# Autodesk Inventor assembly: focus_m12_n12_f=6.0lam_to_14.0lam_step=2.0lam_assembly
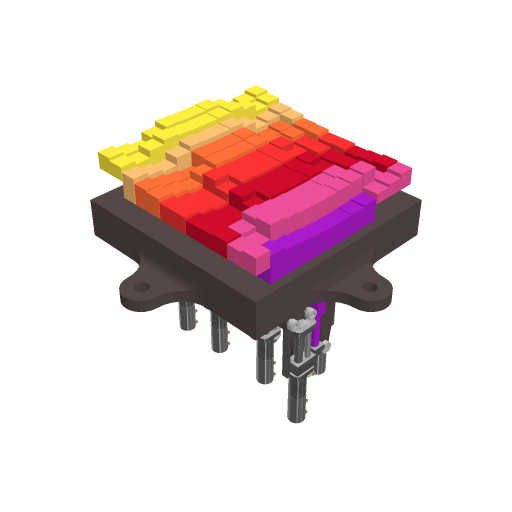
[picture p0: Inventor's stored thumbnail of the model, 512x512]
Saved by Autodesk Inventor 2023 (Build 270158000, 158)
## iProperties
Created: 2022-08-15
Part Number: focus_m12_n12_f=6.0lam_to_14.0lam_step=2.0lam_assembly
Document SubType Name: Assembly
Designer: James
Author: James
## Documents named in this file (14)
- C:\Users\James\OneDrive - University College London\Activation of Metasurface\Ben Motors\SSM_assembly\focus_m12_n12_f=6.0lam_to_14.0lam_step=2.0lam_assembly.iam
- C:\Users\James\OneDrive - University College London\Activation of Metasurface\Ben Motors\SSM_assembly\seg_1.ipt
- C:\Users\James\OneDrive - University College London\Activation of Metasurface\Ben Motors\SSM_assembly\seg_2.ipt
- C:\Users\James\OneDrive - University College London\Activation of Metasurface\Ben Motors\SSM_assembly\seg_3.ipt
- C:\Users\James\OneDrive - University College London\Activation of Metasurface\Ben Motors\SSM_assembly\seg_4.ipt
- C:\Users\James\OneDrive - University College London\Activation of Metasurface\Ben Motors\SSM_assembly\seg_5.ipt
- C:\Users\James\OneDrive - University College London\Activation of Metasurface\Ben Motors\SSM_assembly\seg_6.ipt
- C:\Users\James\OneDrive - University College London\Activation of Metasurface\Ben Motors\SSM_assembly\seg_7.ipt
- C:\Users\James\OneDrive - University College London\Activation of Metasurface\Ben Motors\SSM_assembly\jig.iam
- C:\Users\James\OneDrive - University College London\Activation of Metasurface\Ben Motors\SSM_assembly\motor_lowest.ipt
- C:\Users\James\OneDrive - University College London\Activation of Metasurface\Ben Motors\SSM_assembly\motor_mid.ipt
- C:\Users\James\OneDrive - University College London\Activation of Metasurface\Ben Motors\SSM_assembly\motor_highest.ipt
- C:\Users\James\OneDrive - University College London\Activation of Metasurface\Ben Motors\SSM_assembly\M1.4 Hex Screw v3.ipt
- C:\Users\James\OneDrive - University College London\Activation of Metasurface\Ben Motors\SSM_assembly\Nut M1.4 v3.ipt
## Components (57 placed, 13 different names)
1. jig:1 [sub-assembly] — Mate:16, Flush:8, Mate:19, Mate:20, Mate:24, Mate:25, Mate:26, Mate:28, Flush:9, Mate:29, Flush:10, Flush:11, Flush:12, Flush:13, Flush:14, Flush:15, Flush:16, Flush:17, Flush:18, Flush:19, Flush:20, Flush:21, Flush:22, Flush:23, Mate:90, Mate:91, Mate:126, Mate:127
2. motor_highest:1 — Mate:28, Flush:10, Flush:17, Mate:45, Mate:46, Mate:47, Mate:48, Mate:49
3. motor_mid:1 — Mate:19, Flush:15, Flush:22, Mate:74, Mate:75, Mate:76, Mate:77, Mate:78, Mate:79
4. motor_mid:2 — Mate:20, Flush:13, Flush:21, Mate:62, Mate:63, Mate:64, Mate:65, Mate:66, Mate:67
5. motor_mid:3 — Mate:24, Flush:14, Flush:19, Mate:68, Mate:69, Mate:70, Mate:71, Mate:72, Mate:73
6. motor_mid:4 — Mate:25, Flush:12, Flush:18, Mate:56, Mate:57, Mate:58, Mate:59, Mate:60, Mate:61
7. motor_mid:5 — Mate:26, Flush:11, Flush:20, Mate:50, Mate:51, Mate:52, Mate:53, Mate:54, Mate:55
8. motor_lowest:1 — Mate:16, Flush:16, Flush:23, Mate:80, Mate:81, Mate:82, Mate:83, Mate:84, Mate:85
9. seg_1:1 — Mate:7, Mate:8, Flush:1, Mate:9
10. seg_2:1 — Mate:6, Mate:10, Mate:14, Flush:7
11. seg_3:1 — Mate:5, Mate:8, Flush:1, Flush:2, Flush:6
12. seg_4:1 — Mate:4, Flush:5, Mate:10, Mate:13, Mate:14
13. seg_5:1 — Mate:3, Flush:2, Mate:9, Flush:3, Flush:4, Flush:5, Mate:11
14. seg_6:1 — Mate:2, Flush:3, Mate:11, Mate:12
15. seg_7:1 — Mate:1, Flush:4, Mate:12, Mate:13
16. M1.4 Hex Screw v3:1 — Mate:45, Mate:88
17. M1.4 Hex Screw v3:2 — Mate:46, Mate:47, Mate:86
18. M1.4 Hex Screw v3:3 — Mate:48, Mate:49, Mate:89
19. M1.4 Hex Screw v3:4 — Mate:50, Mate:53, Mate:94
20. M1.4 Hex Screw v3:5 — Mate:51, Mate:54, Mate:93
21. M1.4 Hex Screw v3:6 — Mate:52, Mate:55, Mate:92
22. M1.4 Hex Screw v3:7 — Mate:56, Mate:60, Mate:98
23. M1.4 Hex Screw v3:8 — Mate:58, Mate:61, Mate:100
24. M1.4 Hex Screw v3:9 — Mate:57, Mate:59, Mate:99
25. M1.4 Hex Screw v3:10 — Mate:62, Mate:65, Mate:104
26. M1.4 Hex Screw v3:11 — Mate:63, Mate:66, Mate:105
27. M1.4 Hex Screw v3:12 — Mate:64, Mate:67, Mate:106
28. M1.4 Hex Screw v3:13 — Mate:69, Mate:73, Mate:111
29. M1.4 Hex Screw v3:14 — Mate:70, Mate:72, Mate:110
30. M1.4 Hex Screw v3:15 — Mate:68, Mate:71, Mate:112
31. M1.4 Hex Screw v3:16 — Mate:76, Mate:77, Mate:117
32. M1.4 Hex Screw v3:17 — Mate:75, Mate:78, Mate:116
33. M1.4 Hex Screw v3:18 — Mate:74, Mate:79, Mate:118
34. M1.4 Hex Screw v3:19 — Mate:82, Mate:83, Mate:123
35. M1.4 Hex Screw v3:20 — Mate:80, Mate:84, Mate:122
36. M1.4 Hex Screw v3:21 — Mate:81, Mate:85, Mate:124
37. Nut M1.4 v3:1 — Mate:86
38. Nut M1.4 v3:2 — Mate:88, Mate:90
39. Nut M1.4 v3:3 — Mate:89, Mate:91
40. Nut M1.4 v3:4 — Mate:92
41. Nut M1.4 v3:5 — Mate:93
42. Nut M1.4 v3:6 — Mate:94
43. Nut M1.4 v3:7 — Mate:98
44. Nut M1.4 v3:8 — Mate:100
45. Nut M1.4 v3:9 — Mate:99
46. Nut M1.4 v3:10 — Mate:104
47. Nut M1.4 v3:11 — Mate:106
48. Nut M1.4 v3:12 — Mate:105
49. Nut M1.4 v3:13 — Mate:112
50. Nut M1.4 v3:14 — Mate:110
51. Nut M1.4 v3:15 — Mate:111
52. Nut M1.4 v3:16 — Mate:116
53. Nut M1.4 v3:17 — Mate:117
54. Nut M1.4 v3:18 — Mate:118
55. Nut M1.4 v3:19 — Mate:122
56. Nut M1.4 v3:20 — Mate:123, Mate:126
57. Nut M1.4 v3:21 — Mate:124, Mate:127
## Relationships (111: Mate 88, Flush 23)
- Mate:1 (4.2875 mm): seg_7:1
- Mate:2 (4.2875 mm): seg_6:1
- Mate:3 (4.2875 mm): seg_5:1
- Mate:4 (4.2875 mm): seg_4:1
- Mate:5 (8.575 mm): seg_3:1
- Mate:6: seg_2:1
- Mate:7 (4.2875 mm): seg_1:1
- Mate:8 (0.2 mm): seg_1:1 ↔ seg_3:1
- Flush:1: seg_1:1 ↔ seg_3:1
- Flush:2: seg_3:1 ↔ seg_5:1
- Mate:9 (0.2 mm): seg_1:1 ↔ seg_5:1
- Flush:3: seg_5:1 ↔ seg_6:1
- Flush:4: seg_5:1 ↔ seg_7:1
- Flush:5: seg_4:1 ↔ seg_5:1
- Mate:10 (0.2 mm): seg_2:1 ↔ seg_4:1
- Mate:11 (0.2 mm): seg_5:1 ↔ seg_6:1
- Mate:12 (0.2 mm): seg_6:1 ↔ seg_7:1
- Mate:13 (0.2 mm): seg_4:1 ↔ seg_7:1
- Mate:14 (0.2 mm): seg_2:1 ↔ seg_4:1
- Flush:6 (-25.625 mm): seg_3:1
- Flush:7 (25.625 mm): seg_2:1
- Mate:16 (8.165 mm): jig:1 ↔ motor_lowest:1
- Flush:8: jig:1
- Mate:19 (8.165 mm): jig:1 ↔ motor_mid:1
- Mate:20 (8.165 mm): jig:1 ↔ motor_mid:2
- Mate:24 (8.165 mm): jig:1 ↔ motor_mid:3
- Mate:25 (8.165 mm): jig:1 ↔ motor_mid:4
- Mate:26 (8.165 mm): jig:1 ↔ motor_mid:5
- Mate:28 (8.165 mm): jig:1 ↔ motor_highest:1
- Flush:9 (-27.825 mm): jig:1
- Mate:29 (-27.825 mm): jig:1
- Flush:10 (5.038 mm): jig:1 ↔ motor_highest:1
- Flush:11 (10.369 mm): jig:1 ↔ motor_mid:5
- Flush:12 (18.001 mm): jig:1 ↔ motor_mid:4
- Flush:13 (25.373 mm): jig:1 ↔ motor_mid:2
- Flush:14 (35.05 mm): jig:1 ↔ motor_mid:3
- Flush:15 (42.625 mm): jig:1 ↔ motor_mid:1
- Flush:16 (50.056 mm): jig:1 ↔ motor_lowest:1
- Flush:17 (18.555 mm): jig:1 ↔ motor_highest:1
- Flush:18 (18.555 mm): jig:1 ↔ motor_mid:4
- Flush:19 (18.555 mm): jig:1 ↔ motor_mid:3
- Flush:20 (18.555 mm): jig:1 ↔ motor_mid:5
- Flush:21 (18.555 mm): jig:1 ↔ motor_mid:2
- Flush:22 (18.555 mm): jig:1 ↔ motor_mid:1
- Flush:23 (14.268 mm): jig:1 ↔ motor_lowest:1
- Mate:45: motor_highest:1 ↔ M1.4 Hex Screw v3:1
- Mate:46: motor_highest:1 ↔ M1.4 Hex Screw v3:2
- Mate:47: motor_highest:1 ↔ M1.4 Hex Screw v3:2
- Mate:48: motor_highest:1 ↔ M1.4 Hex Screw v3:3
- Mate:49: motor_highest:1 ↔ M1.4 Hex Screw v3:3
- Mate:50: motor_mid:5 ↔ M1.4 Hex Screw v3:4
- Mate:51: motor_mid:5 ↔ M1.4 Hex Screw v3:5
- Mate:52: motor_mid:5 ↔ M1.4 Hex Screw v3:6
- Mate:53: motor_mid:5 ↔ M1.4 Hex Screw v3:4
- Mate:54: motor_mid:5 ↔ M1.4 Hex Screw v3:5
- Mate:55: motor_mid:5 ↔ M1.4 Hex Screw v3:6
- Mate:56: motor_mid:4 ↔ M1.4 Hex Screw v3:7
- Mate:57: motor_mid:4 ↔ M1.4 Hex Screw v3:9
- Mate:58: motor_mid:4 ↔ M1.4 Hex Screw v3:8
- Mate:59: motor_mid:4 ↔ M1.4 Hex Screw v3:9
- Mate:60: motor_mid:4 ↔ M1.4 Hex Screw v3:7
- Mate:61: motor_mid:4 ↔ M1.4 Hex Screw v3:8
- Mate:62: motor_mid:2 ↔ M1.4 Hex Screw v3:10
- Mate:63: motor_mid:2 ↔ M1.4 Hex Screw v3:11
- Mate:64: motor_mid:2 ↔ M1.4 Hex Screw v3:12
- Mate:65: motor_mid:2 ↔ M1.4 Hex Screw v3:10
- Mate:66: motor_mid:2 ↔ M1.4 Hex Screw v3:11
- Mate:67: motor_mid:2 ↔ M1.4 Hex Screw v3:12
- Mate:68: motor_mid:3 ↔ M1.4 Hex Screw v3:15
- Mate:69: motor_mid:3 ↔ M1.4 Hex Screw v3:13
- Mate:70: motor_mid:3 ↔ M1.4 Hex Screw v3:14
- Mate:71: motor_mid:3 ↔ M1.4 Hex Screw v3:15
- Mate:72: motor_mid:3 ↔ M1.4 Hex Screw v3:14
- Mate:73: motor_mid:3 ↔ M1.4 Hex Screw v3:13
- Mate:74: motor_mid:1 ↔ M1.4 Hex Screw v3:18
- Mate:75: motor_mid:1 ↔ M1.4 Hex Screw v3:17
- Mate:76: motor_mid:1 ↔ M1.4 Hex Screw v3:16
- Mate:77: motor_mid:1 ↔ M1.4 Hex Screw v3:16
- Mate:78: motor_mid:1 ↔ M1.4 Hex Screw v3:17
- Mate:79: motor_mid:1 ↔ M1.4 Hex Screw v3:18
- Mate:80: motor_lowest:1 ↔ M1.4 Hex Screw v3:20
- Mate:81: motor_lowest:1 ↔ M1.4 Hex Screw v3:21
- Mate:82: motor_lowest:1 ↔ M1.4 Hex Screw v3:19
- Mate:83: motor_lowest:1 ↔ M1.4 Hex Screw v3:19
- Mate:84: motor_lowest:1 ↔ M1.4 Hex Screw v3:20
- Mate:85: motor_lowest:1 ↔ M1.4 Hex Screw v3:21
- Mate:86: M1.4 Hex Screw v3:2 ↔ Nut M1.4 v3:1
- Mate:88: M1.4 Hex Screw v3:1 ↔ Nut M1.4 v3:2
- Mate:89: M1.4 Hex Screw v3:3 ↔ Nut M1.4 v3:3
- Mate:90: jig:1 ↔ Nut M1.4 v3:2
- Mate:91: jig:1 ↔ Nut M1.4 v3:3
- Mate:92: M1.4 Hex Screw v3:6 ↔ Nut M1.4 v3:4
- Mate:93: M1.4 Hex Screw v3:5 ↔ Nut M1.4 v3:5
- Mate:94: M1.4 Hex Screw v3:4 ↔ Nut M1.4 v3:6
- Mate:98: M1.4 Hex Screw v3:7 ↔ Nut M1.4 v3:7
- Mate:99: M1.4 Hex Screw v3:9 ↔ Nut M1.4 v3:9
- Mate:100: M1.4 Hex Screw v3:8 ↔ Nut M1.4 v3:8
- Mate:104: M1.4 Hex Screw v3:10 ↔ Nut M1.4 v3:10
- Mate:105: M1.4 Hex Screw v3:11 ↔ Nut M1.4 v3:12
- Mate:106: M1.4 Hex Screw v3:12 ↔ Nut M1.4 v3:11
- Mate:110: M1.4 Hex Screw v3:14 ↔ Nut M1.4 v3:14
- Mate:111: M1.4 Hex Screw v3:13 ↔ Nut M1.4 v3:15
- Mate:112: M1.4 Hex Screw v3:15 ↔ Nut M1.4 v3:13
- Mate:116: M1.4 Hex Screw v3:17 ↔ Nut M1.4 v3:16
- Mate:117: M1.4 Hex Screw v3:16 ↔ Nut M1.4 v3:17
- Mate:118: M1.4 Hex Screw v3:18 ↔ Nut M1.4 v3:18
- Mate:122: M1.4 Hex Screw v3:20 ↔ Nut M1.4 v3:19
- Mate:123: M1.4 Hex Screw v3:19 ↔ Nut M1.4 v3:20
- Mate:124: M1.4 Hex Screw v3:21 ↔ Nut M1.4 v3:21
- Mate:126: jig:1 ↔ Nut M1.4 v3:20
- Mate:127: jig:1 ↔ Nut M1.4 v3:21
